# Autodesk Inventor assembly: 3030bracket_MIR_MIR1
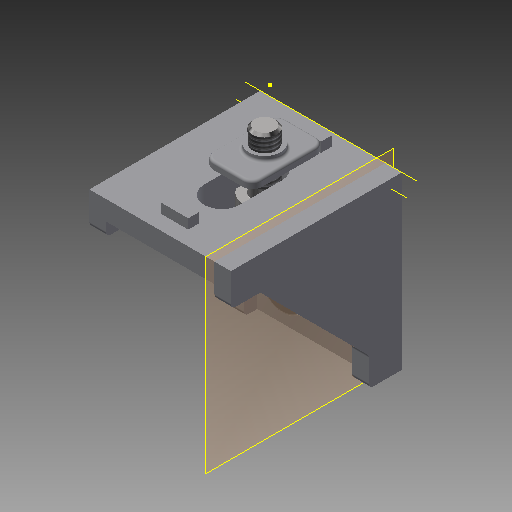
[picture p0: Inventor's stored thumbnail of the model, 512x512]
Saved by Autodesk Inventor 2018 (Build 220112000, 112)
## iProperties
Created: 2016-07-21
Part Number: 3030bracket_MIR_MIR1
Document SubType Name: Assembly
Designer: User
Author: User
## Documents named in this file (5)
- C:\Users\Dan\OneDrive\SL-Inventor\The Beast v1.2 PackandGo\Workspaces\Workspace\3030bracket_MIR_MIR1.iam
- C:\Users\Dan\OneDrive\SL-Inventor\The Beast v1.2 PackandGo\Workspaces\Workspace\30mm Bracket_CPY_MIR2_MIR1.ipt
- C:\Users\Dan\OneDrive\SL-Inventor\The Beast v1.2 PackandGo\Workspaces\Workspace\en-US\ANSI B18.3.1M(6)\ANSI B18.3.1M - M5x0.8 x 12(1).ipt
- C:\Users\Dan\OneDrive\SL-Inventor\The Beast v1.2 PackandGo\Workspaces\Workspace\en-US\ANSI B18.3.1M(6)\ANSI B18.3.1M - M6x1 x 10(1).ipt
- C:\Users\Dan\OneDrive\SL-Inventor\The Beast v1.2 PackandGo\Workspaces\Workspace\M5 Tee Nut_MIR_MIR_MIR_MIR1.ipt
## Components (5 placed, 4 different names)
1. 30mm Bracket_CPY_MIR2_MIR1:1 — Mate:1, Mate:2, Insert:1
2. Forged Socket Head Cap Screw - Metric M5x0.8 x 12:1 — Mate:1, Mate:2, Mate:3
3. Forged Socket Head Cap Screw - Metric M6x1 x 10:1 — Insert:1, Mate:4
4. M5 Tee Nut_MIR_MIR_MIR_MIR1:1 — Mate:3
5. M5 Tee Nut_MIR_MIR_MIR_MIR1:2 — Mate:4
## Relationships (5: Mate 4, Insert 1)
- Mate:1: 30mm Bracket_CPY_MIR2_MIR1:1 ↔ Forged Socket Head Cap Screw - Metric M5x0.8 x 12:1
- Mate:2: 30mm Bracket_CPY_MIR2_MIR1:1 ↔ Forged Socket Head Cap Screw - Metric M5x0.8 x 12:1
- Insert:1: 30mm Bracket_CPY_MIR2_MIR1:1 ↔ Forged Socket Head Cap Screw - Metric M6x1 x 10:1
- Mate:3: Forged Socket Head Cap Screw - Metric M5x0.8 x 12:1 ↔ M5 Tee Nut_MIR_MIR_MIR_MIR1:1
- Mate:4: Forged Socket Head Cap Screw - Metric M6x1 x 10:1 ↔ M5 Tee Nut_MIR_MIR_MIR_MIR1:2
